# Autodesk Inventor assembly: 9P 18T Sprocket, No Insert_MIR
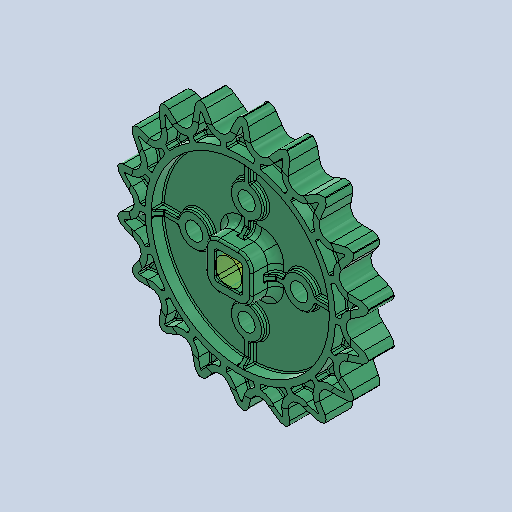
[picture p0: Inventor's stored thumbnail of the model, 512x512]
Saved by Autodesk Inventor 2023.2 (Build 272271030, 271C)
## iProperties
Created: 2022-08-02
Part Number: 9P 18T Sprocket, No Insert_MIR
Document SubType Name: Assembly
Designer: Main Account
Author: ylu12
## Documents named in this file (2)
- C:\Users\Main Account\InventorProjects\VEX\Projects\SpinUpRobots\Catapult\Mirror Dump\9P 18T Sprocket, No Insert_MIR.iam
- C:\Users\Main Account\InventorProjects\VEX\Projects\SpinUpRobots\Catapult\Mirror Dump\9P 18T Sprocket, No Insert_MIR.ipt
## Components (1 placed, 1 different names)
1. 9P 18T Sprocket, No Insert_MIR:1 — Mate:10, Mate:9, Flush:5
## Relationships (3: Mate 2, Flush 1)
- Mate:10: 9P 18T Sprocket, No Insert_MIR:1
- Mate:9: 9P 18T Sprocket, No Insert_MIR:1
- Flush:5: 9P 18T Sprocket, No Insert_MIR:1
